# Autodesk Inventor assembly: Сборочка
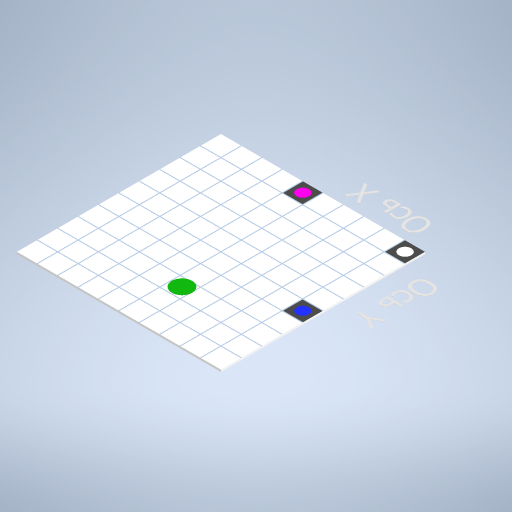
[picture p0: Inventor's stored thumbnail of the model, 512x512]
Saved by Autodesk Inventor 2023.2 (Build 272271030, 271C)
## iProperties
Created: 2025-05-13
Part Number: Сборочка
Document SubType Name: Assembly
Designer: e5470
Author: e5470
## Documents named in this file (3)
- C:\Users\e5470\Desktop\Учёба\2 сем\питон\projekt\Сборочка.iam
- C:\Users\e5470\Desktop\Учёба\2 сем\питон\projekt\деталь.ipt
- C:\Users\e5470\Desktop\Учёба\2 сем\питон\projekt\поле.ipt
## Components (2 placed, 2 different names)
1. деталь:1 — Совмещение:1
2. поле:1 — Совмещение:1
## Relationships (1: Mate 1)
- Совмещение:1 [Mate]: деталь:1 ↔ поле:1
